# Autodesk Inventor assembly: Assembly1
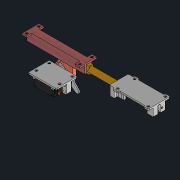
[picture p0: Inventor's stored thumbnail of the model, 180x180]
Saved by Autodesk Inventor 2022.2 (Build 262287010, 287A)
## iProperties
Created: 2022-06-04
Part Number: Assembly1
Document SubType Name: Assembly
Designer: frede
Author: frede
## Documents named in this file (10)
- F:\Documents\Git_Projects\DigCow\CAD\HydrolicDriver.iam
- F:\Documents\Git_Projects\DigCow\CAD\Servo_Motor_MG996R.ipt
- F:\Documents\Git_Projects\DigCow\CAD\Rack222.ipt
- F:\Documents\Git_Projects\DigCow\CAD\Pinion222.ipt
- F:\Documents\Git_Projects\DigCow\CAD\Syringe.ipt
- F:\Documents\Git_Projects\DigCow\CAD\RackSlider.ipt
- C:\Users\sebth\Documents\Inventor\Content Center Files\R2022\en-US\DIN 912\DIN 912 - M3 x 0.5 x 10 x 8.75.ipt
- F:\Documents\Git_Projects\DigCow\CAD\MotorCasingSmall.ipt
- F:\Documents\Git_Projects\DigCow\CAD\SyringeCasing.ipt
- F:\Documents\Git_Projects\DigCow\CAD\NyArm.ipt
## Components (9 placed, 9 different names)
1. Servo_Motor_MG996R:1 — Angle:2, Flush:2, Angle:3, Flush:3, Flush:4, Insert:4, Insert:6, Mate:3, Mate:5
2. NyArm:1 — Insert:4, Insert:6, Flush:7, Mate:4
3. Pinion222:1 — Rotation/Translation:1, Mate:3, Flush:7, Insert:7, Mate:4, Rotation:1, Flush:8
4. DIN 912 - replaced by DIN EN ISO 4762 M3 x 10:1 — Insert:7, Rotation:1
5. Rack222:1 — Angle:2, Flush:2, Rotation/Translation:1, Insert:2, Mate:1, Mate:2, Flush:6, Flush:8
6. Syringe:1 — Insert:2, Angle:3, Mate:5
7. RackSlider:1 — Mate:1, Mate:2, Flush:3, Flush:5, Flush:6
8. MotorCasingSmall:1 — Flush:4
9. SyringeCasing:1 — Flush:5
## Relationships (20: Flush 7, Mate 5, Insert 4, Angle 2, RelateRotateTranslate 1, RelateRotation 1)
- Angle:2 (0 deg): Servo_Motor_MG996R:1 ↔ Rack222:1
- Flush:2 (32.6 mm): Servo_Motor_MG996R:1 ↔ Rack222:1
- Rotation/Translation:1 [RelateRotateTranslate] (183 mm): Pinion222:1 ↔ Rack222:1
- Insert:2 (1.5 mm): Rack222:1 ↔ Syringe:1
- Angle:3 (0 deg): Servo_Motor_MG996R:1 ↔ Syringe:1
- Mate:1 (0.1 mm): Rack222:1 ↔ RackSlider:1
- Mate:2 (0.5 mm): Rack222:1 ↔ RackSlider:1
- Flush:3 (53 mm): Servo_Motor_MG996R:1 ↔ RackSlider:1
- Flush:4: Servo_Motor_MG996R:1 ↔ MotorCasingSmall:1
- Flush:5: RackSlider:1 ↔ SyringeCasing:1
- Insert:4: Servo_Motor_MG996R:1 ↔ NyArm:1
- Flush:6 (30 mm): Rack222:1 ↔ RackSlider:1
- Insert:6: Servo_Motor_MG996R:1 ↔ NyArm:1
- Mate:3: Servo_Motor_MG996R:1 ↔ Pinion222:1
- Flush:7: NyArm:1 ↔ Pinion222:1
- Insert:7: Pinion222:1 ↔ DIN 912 - replaced by DIN EN ISO 4762 M3 x 10:1
- Mate:4: NyArm:1 ↔ Pinion222:1
- Rotation:1 [RelateRotation] (1 ul): Pinion222:1 ↔ DIN 912 - replaced by DIN EN ISO 4762 M3 x 10:1
- Flush:8: Pinion222:1 ↔ Rack222:1
- Mate:5 (94.5 mm): Servo_Motor_MG996R:1 ↔ Syringe:1
